# Autodesk Inventor assembly: 200-60-DIFFERENTIAL-CONNECTOR-02
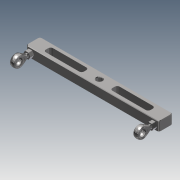
[picture p0: Inventor's stored thumbnail of the model, 180x180]
Saved by Autodesk Inventor 2018.2 (Build 222227000, 227)
## iProperties
Manager: feesmrt
Company: FRANC0R
Created: 2017-12-19
Part Number: 200-60-DIFFERENTIAL-CONNECTOR-02
Project: Rescue Robot
Cost Center: -
Material: Generisch
Document SubType Name: Assembly
Designer: feesmrt
Engineer: feesmrt
Authority: feesmrt
Description: Differential Connector Arm
Stock Number: 200-60-DIFFERENTIAL-CONNECTOR-02
Subject: Rescue Robot
Author: feesmrt
Revision Number: 1
Title: Differential Connector Arm
## Documents named in this file (4)
- D:\Programmierung\FRANC0R\CAD\02-Rocker-Bogie-Robot\200-ROCKER-BOGIE\200-60-DIFFERENTIAL\200-60-DIFFERENTIAL-CONNECTOR-02.iam
- D:\Programmierung\FRANC0R\CAD\02-Rocker-Bogie-Robot\200-ROCKER-BOGIE\200-60-DIFFERENTIAL\200-60-DIFFERENTIAL-CONNECTOR-01.ipt
- D:\Programmierung\FRANC0R\CAD\02-Rocker-Bogie-Robot\900-COMPONENTS\900-70-ANGLE-JOINTS\900-70-ANGLE-JOINT-DIN648-M8-1.ipt
- D:\Programmierung\FRANC0R\CAD\02-Rocker-Bogie-Robot\900-COMPONENTS\900-41-NUTS\900-41-NUTS-ISO4035-M8.ipt
## Components (7 placed, 3 different names)
1. 200-60-DIFFERENTIAL-CONNECTOR-01:1 — Passend:1, Passend:2, Passend:3, Passend:4, Winkel:1, Winkel:2, Passend:7, Passend:11
2. 900-70-ANGLE-JOINT-DIN648-M8-1:1 — Passend:1, Passend:4, Winkel:1, Passend:5, Passend:6
3. 900-70-ANGLE-JOINT-DIN648-M8-1:2 — Passend:2, Passend:3, Winkel:2, Passend:9, Passend:10
4. 900-41-NUTS-ISO4035-M8:1 — Passend:6, Passend:8
5. 900-41-NUTS-ISO4035-M8:2 — Passend:5, Passend:7, Passend:8
6. 900-41-NUTS-ISO4035-M8:3 — Passend:10, Passend:11, Passend:12
7. 900-41-NUTS-ISO4035-M8:4 — Passend:9, Passend:12
## Relationships (14: Mate 12, Angle 2)
- Passend:1 [Mate]: 200-60-DIFFERENTIAL-CONNECTOR-01:1 ↔ 900-70-ANGLE-JOINT-DIN648-M8-1:1
- Passend:2 [Mate]: 200-60-DIFFERENTIAL-CONNECTOR-01:1 ↔ 900-70-ANGLE-JOINT-DIN648-M8-1:2
- Passend:3 [Mate] (10.48 mm): 200-60-DIFFERENTIAL-CONNECTOR-01:1 ↔ 900-70-ANGLE-JOINT-DIN648-M8-1:2
- Passend:4 [Mate] (10.48 mm): 200-60-DIFFERENTIAL-CONNECTOR-01:1 ↔ 900-70-ANGLE-JOINT-DIN648-M8-1:1
- Winkel:1 [Angle] (90 deg): 200-60-DIFFERENTIAL-CONNECTOR-01:1 ↔ 900-70-ANGLE-JOINT-DIN648-M8-1:1
- Winkel:2 [Angle] (90 deg): 200-60-DIFFERENTIAL-CONNECTOR-01:1 ↔ 900-70-ANGLE-JOINT-DIN648-M8-1:2
- Passend:5 [Mate]: 900-70-ANGLE-JOINT-DIN648-M8-1:1 ↔ 900-41-NUTS-ISO4035-M8:2
- Passend:6 [Mate]: 900-70-ANGLE-JOINT-DIN648-M8-1:1 ↔ 900-41-NUTS-ISO4035-M8:1
- Passend:7 [Mate]: 200-60-DIFFERENTIAL-CONNECTOR-01:1 ↔ 900-41-NUTS-ISO4035-M8:2
- Passend:8 [Mate]: 900-41-NUTS-ISO4035-M8:1 ↔ 900-41-NUTS-ISO4035-M8:2
- Passend:9 [Mate]: 900-70-ANGLE-JOINT-DIN648-M8-1:2 ↔ 900-41-NUTS-ISO4035-M8:4
- Passend:10 [Mate]: 900-70-ANGLE-JOINT-DIN648-M8-1:2 ↔ 900-41-NUTS-ISO4035-M8:3
- Passend:11 [Mate]: 200-60-DIFFERENTIAL-CONNECTOR-01:1 ↔ 900-41-NUTS-ISO4035-M8:3
- Passend:12 [Mate]: 900-41-NUTS-ISO4035-M8:3 ↔ 900-41-NUTS-ISO4035-M8:4
